# Autodesk Inventor assembly: arm
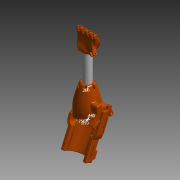
[picture p0: Inventor's stored thumbnail of the model, 180x180]
Saved by Autodesk Inventor 2015 (Build 190159000, 159)
## iProperties
Created: 2014-05-06
Part Number: arm
Document SubType Name: Assembly
Designer: Jascha
Author: Jascha
## Documents named in this file (7)
- C:\Users\Jascha\Dropbox\enable\transradial arm\RIT arm\v0.43\arm.iam
- C:\Users\Jascha\Dropbox\enable\transradial arm\RIT arm\v0.43\pipe.ipt
- C:\Users\Jascha\Dropbox\enable\transradial arm\RIT arm\v0.43\palm.ipt
- C:\Users\Jascha\Dropbox\enable\transradial arm\derek black\v0.3\forearm swivel adapter.ipt
- C:\Users\Jascha\Dropbox\enable\transradial arm\RIT arm\v0.43\forearm cup.ipt
- C:\Users\Jascha\Dropbox\enable\transradial arm\RIT arm\v0.43\triceps cuff.ipt
- C:\Users\Jascha\Dropbox\enable\transradial arm\RIT arm\v0.43\tensioners.ipt
## Components (10 placed, 6 different names)
1. pipe:1
2. palm:1 — Flush:1, Flush:4
3. forearm swivel adapter:1 — Flush:2, Flush:3
4. forearm cup:1 — Flush:3, Mate:1, Mate:2, Flush:8, Flush:9, Mate:5
5. triceps cuff:1 — Flush:8, Mate:4, Mate:6, Flush:10
6. tensioners:1 — Mate:6, Flush:10
7. tensioners:2
8. tensioners:3
9. tensioners:4
10. tensioners:5
## Component patterns: (5 elements, first: tensioners:1)
## Relationships (13: Flush 7, Mate 6)
- Flush:1 (-50.8 mm): palm:1
- Flush:2 (-57.15 mm): forearm swivel adapter:1
- Flush:3: forearm swivel adapter:1 ↔ forearm cup:1
- Flush:4 (-4 mm): palm:1
- Mate:1: forearm cup:1
- Mate:2: forearm cup:1
- Mate:3
- Flush:8: forearm cup:1 ↔ triceps cuff:1
- Mate:4: triceps cuff:1
- Flush:9: forearm cup:1
- Mate:5: forearm cup:1
- Mate:6: triceps cuff:1 ↔ tensioners:1
- Flush:10 (5 mm): triceps cuff:1 ↔ tensioners:1
